# Autodesk Inventor assembly: Ensamblaje1
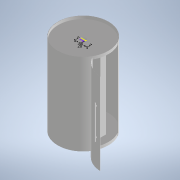
[picture p0: Inventor's stored thumbnail of the model, 180x180]
Saved by Autodesk Inventor 2021 (Build 250183000, 183)
## iProperties
Created: 2021-11-08
Part Number: Ensamblaje1
Document SubType Name: Assembly
Designer: arthu
Author: arthu
## Documents named in this file (6)
- C:\Users\arthu\OneDrive\Escritorio\TersusMax\ir_cafe\Ensamblaje1.iam
- C:\Users\arthu\OneDrive\Escritorio\TersusMax\ir_cafe\tapa_tambor.ipt
- C:\Users\arthu\OneDrive\Escritorio\TersusMax\ir_cafe\tambor.ipt
- C:\Users\arthu\OneDrive\Escritorio\TersusMax\ir_cafe\ventana_tambor.ipt
- C:\Users\arthu\OneDrive\Escritorio\TersusMax\ir_cafe\ir+marco.iam
- C:\Users\arthu\OneDrive\Escritorio\TersusMax\ir_cafe\tapa_marco.ipt
## Components (6 placed, 5 different names)
1. tapa_tambor:1 — Rígido:1
2. tapa_tambor:2 — De rotación:1, Rígido:2
3. tambor:1 — De rotación:1, Rígido:1, De rotación:2
4. ventana_tambor:1 — De rotación:2
5. ir+marco:1 [sub-assembly] — Rígido:2, De rotación:3
6. tapa_marco:1 — De rotación:3
## Relationships (5: RevoluteJoint 3, WeldJoint 2)
- De rotación:1 [RevoluteJoint]: tapa_tambor:2 ↔ tambor:1
- Rígido:1 [WeldJoint]: tapa_tambor:1 ↔ tambor:1
- De rotación:2 [RevoluteJoint]: tambor:1 ↔ ventana_tambor:1
- Rígido:2 [WeldJoint] (-17.5 mm): tapa_tambor:2 ↔ ir+marco:1
- De rotación:3 [RevoluteJoint]: ir+marco:1 ↔ tapa_marco:1
